# Autodesk Inventor assembly: Real assembly
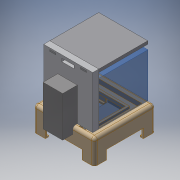
[picture p0: Inventor's stored thumbnail of the model, 180x180]
Saved by Autodesk Inventor 2019 (Build 230136000, 136)
## iProperties
Created: 2016-08-06
Part Number: Real assembly
Document SubType Name: Assembly
Designer: Jorian Brusind
Author: Jorian Brusind
## Documents named in this file (7)
- C:\Users\Jorian Brusind\Documents\GitHub\PersonalProjects\Automated Terrarium Project\Inventor Files\V1\Real assembly.iam
- C:\Users\Jorian Brusind\Documents\GitHub\PersonalProjects\Automated Terrarium Project\Inventor Files\V1\model for case.ipt
- C:\Users\Jorian Brusind\Documents\GitHub\PersonalProjects\Automated Terrarium Project\Inventor Files\V1\back.ipt
- C:\Users\Jorian Brusind\Documents\GitHub\PersonalProjects\Automated Terrarium Project\Inventor Files\V1\top.ipt
- C:\Users\Jorian Brusind\Documents\GitHub\PersonalProjects\Automated Terrarium Project\Inventor Files\V1\Motor.ipt
- C:\Users\Jorian Brusind\Documents\GitHub\PersonalProjects\Automated Terrarium Project\Inventor Files\V1\Part2.ipt
- C:\Users\Jorian Brusind\Documents\GitHub\PersonalProjects\Automated Terrarium Project\Inventor Files\V1\arduinocase.ipt
## Components (6 placed, 6 different names)
1. model for case:1 — Mate:1, Flush:2, Flush:6, Mate:9, Flush:7
2. back:1 — Mate:1, Flush:2, Flush:3, Mate:2, Flush:4, Mate:3, Flush:5, Mate:6
3. top:1 — Flush:3, Mate:2, Flush:4
4. Motor:1 — Mate:3, Flush:5
5. Part2:1 — Mate:6, Mate:9
6. arduinocase:1 — Flush:6, Flush:7
## Relationships (11: Flush 6, Mate 5)
- Mate:1: model for case:1 ↔ back:1
- Flush:2 (12.7 mm): model for case:1 ↔ back:1
- Flush:3: back:1 ↔ top:1
- Mate:2: back:1 ↔ top:1
- Flush:4: back:1 ↔ top:1
- Mate:3: back:1 ↔ Motor:1
- Flush:5 (31.75 mm): back:1 ↔ Motor:1
- Mate:6: back:1 ↔ Part2:1
- Flush:6: model for case:1 ↔ arduinocase:1
- Mate:9: model for case:1 ↔ Part2:1
- Flush:7: model for case:1 ↔ arduinocase:1
